# Autodesk Inventor assembly: MINI_MRI_Screw_lids
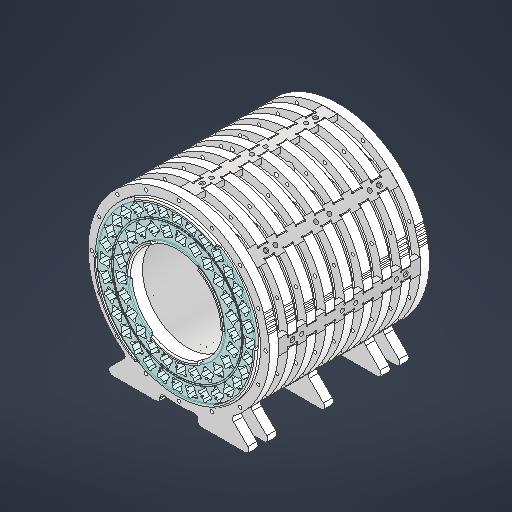
[picture p0: Inventor's stored thumbnail of the model, 512x512]
Saved by Autodesk Inventor 2026.1 (Build 301233020, 233B)
## iProperties
Created: 2025-11-12
Part Number: MINI_MRI_Screw_lids
Document SubType Name: Assembly
Designer: Carla Fernandez
Author: Carla Fernandez
## Documents named in this file (11)
- C:\Users\Carla Fernandez\Documents\GitHub\OSII_MINI_V2\CAD MODELS_screw_on\MINI_MRI_Screw_lids.iam
- C:\Users\Carla Fernandez\Documents\GitHub\OSII_MINI_V2\CAD MODELS_screw_on\Ring_0.ipt
- C:\Users\Carla Fernandez\Documents\GitHub\OSII_MINI_V2\CAD MODELS_screw_on\Ring_1.ipt
- C:\Users\Carla Fernandez\Documents\GitHub\OSII_MINI_V2\CAD MODELS_screw_on\Ring_2.ipt
- C:\Users\Carla Fernandez\Documents\GitHub\OSII_MINI_V2\CAD MODELS_screw_on\Ring_3.ipt
- C:\Users\Carla Fernandez\Documents\GitHub\OSII_MINI_V2\CAD MODELS_screw_on\Ring_4.ipt
- C:\Users\Carla Fernandez\Documents\GitHub\OSII_MINI_V2\CAD MODELS_screw_on\Locating_bar_V2.ipt
- C:\Users\Carla Fernandez\Documents\GitHub\OSII_MINI_V2\CAD MODELS_screw_on\Lid_A.ipt
- C:\Users\Carla Fernandez\Documents\GitHub\OSII_MINI_V2\CAD MODELS_screw_on\Lid_B.ipt
- C:\Users\Carla Fernandez\Documents\GitHub\OSII_MINI_V2\CAD MODELS_screw_on\Gradient_Coil.ipt
- C:\Users\Carla Fernandez\Documents\GitHub\OSII_MINI_V2\CAD MODELS_screw_on\Gradient_positioner.ipt
## Components (28 placed, 10 different names)
1. Ring_0:1 — Flush:1, Flush:2, Flush:3, Flush:4, Flush:5, Flush:6, Flush:7, Flush:8, Flush:9, Flush:10, Flush:11, Flush:12, Flush:13, Flush:14, Flush:15, Flush:16, Flush:17, Flush:18, Flush:19, Flush:20, Mate:1, Flush:21, Flush:22, Flush:24, Flush:28, Angle:33, Mate:2, Mate:3, Mate:6, Flush:32, Flush:34, Mate:7, Mate:8
2. Ring_1:1 — Flush:4, Flush:12, Flush:24, Flush:25
3. Ring_1:2 — Flush:5, Flush:13, Flush:28, Flush:29
4. Ring_2:1 — Flush:6, Flush:14, Flush:25, Flush:26
5. Ring_2:2 — Flush:7, Flush:15, Flush:29, Flush:30
6. Ring_3:1 — Flush:8, Flush:16, Flush:17, Flush:30, Flush:31
7. Ring_3:2 — Flush:9, Flush:18, Flush:26, Flush:27
8. Ring_4:1 — Flush:10, Flush:19, Flush:27, Mate:4, Mate:5
9. Ring_4:2 — Flush:11, Flush:20, Flush:31
10. Gradient_Coil:1 — Mate:6, Flush:32, Flush:33
11. Gradient_positioner:1 — Flush:34, Mate:7, Mate:8
12. Locating_bar_V2:1 — Mate:1, Flush:21, Flush:23
13. Locating_bar_V2:2
14. Locating_bar_V2:3
15. Locating_bar_V2:4
16. Locating_bar_V2:5
17. Locating_bar_V2:6
18. Locating_bar_V2:7
19. Locating_bar_V2:8
20. Lid_A:1 — Angle:33, Mate:2, Mate:3
21. Lid_A:2
22. Lid_A:3
23. Lid_A:4
24. Lid_A:5
25. Lid_A:6
26. Lid_A:7
27. Lid_B:1 — Angle:34, Mate:4, Mate:5
28. Lid_B:2
## Component patterns: (8 elements, first: Locating_bar_V2:1), (7 elements, first: Lid_A:1), (2 elements, first: Lid_B:1)
## Relationships (44: Flush 34, Mate 8, Angle 2)
- Flush:1: Ring_0:1
- Flush:2: Ring_0:1
- Flush:3: Ring_0:1
- Flush:4: Ring_0:1 ↔ Ring_1:1
- Flush:5: Ring_0:1 ↔ Ring_1:2
- Flush:6: Ring_0:1 ↔ Ring_2:1
- Flush:7: Ring_0:1 ↔ Ring_2:2
- Flush:8: Ring_0:1 ↔ Ring_3:1
- Flush:9: Ring_0:1 ↔ Ring_3:2
- Flush:10: Ring_0:1 ↔ Ring_4:1
- Flush:11: Ring_0:1 ↔ Ring_4:2
- Flush:12: Ring_0:1 ↔ Ring_1:1
- Flush:13: Ring_0:1 ↔ Ring_1:2
- Flush:14: Ring_0:1 ↔ Ring_2:1
- Flush:15: Ring_0:1 ↔ Ring_2:2
- Flush:16: Ring_0:1 ↔ Ring_3:1
- Flush:17: Ring_0:1 ↔ Ring_3:1
- Flush:18: Ring_0:1 ↔ Ring_3:2
- Flush:19: Ring_0:1 ↔ Ring_4:1
- Flush:20: Ring_0:1 ↔ Ring_4:2
- Mate:1: Ring_0:1 ↔ Locating_bar_V2:1
- Flush:21: Ring_0:1 ↔ Locating_bar_V2:1
- Flush:22 (-6 mm): Ring_0:1
- Flush:23: Locating_bar_V2:1
- Flush:24 (25 mm): Ring_0:1 ↔ Ring_1:1
- Flush:25 (25 mm): Ring_1:1 ↔ Ring_2:1
- Flush:26 (25 mm): Ring_2:1 ↔ Ring_3:2
- Flush:27 (25 mm): Ring_3:2 ↔ Ring_4:1
- Flush:28 (25 mm): Ring_0:1 ↔ Ring_1:2
- Flush:29 (-25 mm): Ring_1:2 ↔ Ring_2:2
- Flush:30 (-25 mm): Ring_2:2 ↔ Ring_3:1
- Flush:31 (-25 mm): Ring_3:1 ↔ Ring_4:2
- Angle:33 (60 deg): Ring_0:1 ↔ Lid_A:1
- Mate:2: Ring_0:1 ↔ Lid_A:1
- Mate:3: Ring_0:1 ↔ Lid_A:1
- Angle:34 (60 deg): Lid_B:1
- Mate:4: Ring_4:1 ↔ Lid_B:1
- Mate:5: Ring_4:1 ↔ Lid_B:1
- Mate:6: Ring_0:1 ↔ Gradient_Coil:1
- Flush:32: Ring_0:1 ↔ Gradient_Coil:1
- Flush:33 (6 mm): Gradient_Coil:1
- Flush:34: Ring_0:1 ↔ Gradient_positioner:1
- Mate:7: Ring_0:1 ↔ Gradient_positioner:1
- Mate:8: Ring_0:1 ↔ Gradient_positioner:1
